# Autodesk Inventor assembly: Inductor Assembly
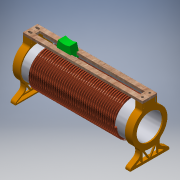
[picture p0: Inventor's stored thumbnail of the model, 180x180]
Saved by Autodesk Inventor 2018 (Build 220112000, 112)
## iProperties
Created: 2017-12-03
Part Number: Inductor Assembly
Document SubType Name: Assembly
Designer: xdlea
Author: xdlea
## Documents named in this file (7)
- D:\Users\Andrew\OneDrive\3D Models\AM Radio\Inductor Assembly.iam
- D:\Users\Andrew\OneDrive\3D Models\AM Radio\Inductor Legs.ipt
- D:\Users\Andrew\OneDrive\3D Models\AM Radio\Inductor.ipt
- D:\Users\Andrew\OneDrive\3D Models\AM Radio\Wood Rail.ipt
- D:\Users\Andrew\OneDrive\3D Models\AM Radio\Wood Rail Selector.ipt
- D:\Users\Andrew\OneDrive\3D Models\AM Radio\Conductive Rail.ipt
- D:\Users\Andrew\OneDrive\3D Models\AM Radio\Wood Rail Selector Conductor.ipt
## Components (8 placed, 6 different names)
1. Inductor Legs:1 — Mate:3, Mate:4, Flush:2, Mate:8, Mate:9, Flush:7
2. Inductor Legs:2 — Mate:5, Mate:6, Flush:3, Mate:10, Mate:11, Mate:12, Mate:13, Flush:9
3. Inductor:1 — Mate:1, Mate:2, Flush:1, Mate:3, Mate:4, Mate:5, Mate:6
4. Wood Rail:1 — Flush:6, Mate:7, Mate:9, Mate:10, Flush:8
5. Wood Rail:2 — Flush:6, Mate:7, Mate:8, Mate:11
6. Wood Rail Selector:1 — Flush:7, Flush:8, Mate:14, Mate:15, Mate:16
7. Conductive Rail:1 — Mate:12, Mate:13, Flush:9
8. Wood Rail Selector Conductor:1 — Mate:14, Mate:15, Mate:16
## Relationships (23: Mate 16, Flush 7)
- Mate:1: Inductor:1
- Mate:2: Inductor:1
- Flush:1: Inductor:1
- Mate:3: Inductor Legs:1 ↔ Inductor:1
- Mate:4: Inductor Legs:1 ↔ Inductor:1
- Mate:5: Inductor Legs:2 ↔ Inductor:1
- Mate:6: Inductor Legs:2 ↔ Inductor:1
- Flush:2: Inductor Legs:1
- Flush:3: Inductor Legs:2
- Flush:6: Wood Rail:1 ↔ Wood Rail:2
- Mate:7: Wood Rail:1 ↔ Wood Rail:2
- Mate:8: Inductor Legs:1 ↔ Wood Rail:2
- Mate:9: Inductor Legs:1 ↔ Wood Rail:1
- Mate:10: Inductor Legs:2 ↔ Wood Rail:1
- Mate:11: Inductor Legs:2 ↔ Wood Rail:2
- Flush:7: Inductor Legs:1 ↔ Wood Rail Selector:1
- Flush:8: Wood Rail:1 ↔ Wood Rail Selector:1
- Mate:12: Inductor Legs:2 ↔ Conductive Rail:1
- Mate:13: Inductor Legs:2 ↔ Conductive Rail:1
- Flush:9: Inductor Legs:2 ↔ Conductive Rail:1
- Mate:14: Wood Rail Selector:1 ↔ Wood Rail Selector Conductor:1
- Mate:15: Wood Rail Selector:1 ↔ Wood Rail Selector Conductor:1
- Mate:16: Wood Rail Selector:1 ↔ Wood Rail Selector Conductor:1
